# Autodesk Inventor assembly: Ring_Finger_assembly_1
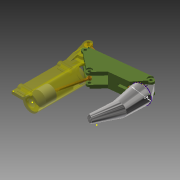
[picture p0: Inventor's stored thumbnail of the model, 180x180]
Saved by Autodesk Inventor 2015 (Build 190159000, 159)
## iProperties
Created: 2016-07-18
Part Number: Ring_Finger_assembly_1
Document SubType Name: Assembly
Designer: Neelotpal Nag
Author: Neelotpal Nag
## Documents named in this file (7)
- D:\NEEL BACKUP\DISA 2016\Fingers 1\Ring_Finger_assembly_1.iam
- D:\NEEL BACKUP\DISA 2016\Fingers 1\Finger_Lower_main_1.ipt
- D:\NEEL BACKUP\DISA 2016\Fingers 1\Restrain_Pin_1.ipt
- D:\NEEL BACKUP\DISA 2016\Fingers 1\Ring_Upper_main_1.ipt
- D:\NEEL BACKUP\DISA 2016\Fingers 1\Shaft_Piston.ipt
- D:\NEEL BACKUP\DISA 2016\Fingers 1\Base_Cylinder_11mm.ipt
- D:\NEEL BACKUP\DISA 2016\Fingers 1\Cylinder_10.5mm.ipt
## Components (6 placed, 6 different names)
1. Finger_Lower_main_1:1 — Mate:6, Mate:9, Mate:10, Mate:15, Mate:16
2. Restrain_Pin_1:1 — Mate:11, Mate:17, Mate:18
3. Ring_Upper_main_1:1 — Mate:9, Mate:10, Mate:11, Mate:17
4. Shaft_Piston:1 — Mate:6, Mate:12, Mate:14
5. Base_Cylinder_11mm:1 — Mate:13, Angle:1, Mate:15, Mate:16, Mate:18
6. Cylinder_10.5mm:1 — Mate:12, Mate:13, Angle:1, Mate:14
## Relationships (12: Mate 11, Angle 1)
- Mate:6: Finger_Lower_main_1:1 ↔ Shaft_Piston:1
- Mate:9: Finger_Lower_main_1:1 ↔ Ring_Upper_main_1:1
- Mate:10: Finger_Lower_main_1:1 ↔ Ring_Upper_main_1:1
- Mate:11: Restrain_Pin_1:1 ↔ Ring_Upper_main_1:1
- Mate:12: Shaft_Piston:1 ↔ Cylinder_10.5mm:1
- Mate:13: Base_Cylinder_11mm:1 ↔ Cylinder_10.5mm:1
- Angle:1 (0 deg): Base_Cylinder_11mm:1 ↔ Cylinder_10.5mm:1
- Mate:14: Shaft_Piston:1 ↔ Cylinder_10.5mm:1
- Mate:15: Finger_Lower_main_1:1 ↔ Base_Cylinder_11mm:1
- Mate:16: Finger_Lower_main_1:1 ↔ Base_Cylinder_11mm:1
- Mate:17 (0.3 mm): Restrain_Pin_1:1 ↔ Ring_Upper_main_1:1
- Mate:18: Restrain_Pin_1:1 ↔ Base_Cylinder_11mm:1
